# Autodesk Inventor assembly: body
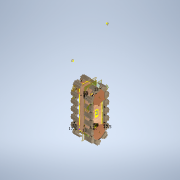
[picture p0: Inventor's stored thumbnail of the model, 180x180]
Saved by Autodesk Inventor 2020 (Build 240168000, 168)
## iProperties
Created: 2020-02-17
Part Number: body
Document SubType Name: Assembly
Designer: erwin
Author: erwin
## Documents named in this file (12)
- D:\GitHub\BeachMaid\platform-2\body.iam
- D:\GitHub\BeachMaid\platform-2\side.ipt
- D:\GitHub\BeachMaid\platform-2\middle.ipt
- D:\GitHub\BeachMaid\platform-2\internal.ipt
- D:\GitHub\BeachMaid\platform-2\cover.ipt
- D:\GitHub\BeachMaid\platform-2\plastic_lip.ipt
- D:\GitHub\BeachMaid\platform-2\spacer_battery_pack.ipt
- D:\GitHub\BeachMaid\platform-2\body\AIP\Tube and Pipe\Cable and Harness\body.Harness1.iam
- D:\GitHub\BeachMaid\platform\vent_cover.ipt
- D:\GitHub\BeachMaid\platform\motor_frontalholder.ipt
- D:\GitHub\BeachMaid\platform\sprocket7.ipt
- D:\GitHub\BeachMaid\platform-2\spacer_chain_link.ipt
## Components (22 placed, 11 different names)
1. side:1 — Flush:1, Flush:2, Flush:4, Rigid:2, Rotational:1, Rotational:4, Rotational:5
2. middle:1 — Flush:1, Flush:2, Mate:1, Flush:3, Flush:5, Flush:6, Flush:7, Flush:8, Mate:4, Mate:5, Planar:1, Planar:3, Planar:4
3. side:2 — Mate:1, Flush:3, Flush:4, Rigid:1, Rotational:2, Rotational:7, Rotational:6
4. internal:1 — Flush:5, Flush:6, Flush:11
5. cover:1 — Flush:7, Flush:8, Flush:9, Flush:10, Flush:11, Mate:2, Flush:12, Mate:3
6. plastic_lip:1 — Flush:9, Flush:10
7. plastic_lip:2 — Mate:2, Flush:12, Mate:3
8. internal:2 — Mate:4, Mate:5
9. spacer_battery_pack:1 — Planar:3
10. spacer_battery_pack:2 — Planar:4
11. spacer_battery_pack:3 — Planar:1
12. Harness1 [sub-assembly]
13. vent_cover:1 — Rigid:2
14. vent_cover:2 — Rigid:1
15. motor_frontalholder:1 — Rotational:2
16. motor_frontalholder:2 — Rotational:1
17. sprocket7:1 — Rotational:6
18. sprocket7:2 — Rotational:4
19. sprocket7:3 — Rotational:5
20. sprocket7:4 — Rotational:7
21. spacer_chain_link:1
22. spacer_chain_link:2
## Relationships (28: Flush 12, RevoluteJoint 6, Mate 5, PlanarJoint 3, WeldJoint 2)
- Flush:1: side:1 ↔ middle:1
- Flush:2: side:1 ↔ middle:1
- Mate:1: middle:1 ↔ side:2
- Flush:3: middle:1 ↔ side:2
- Flush:4: side:1 ↔ side:2
- Flush:5: middle:1 ↔ internal:1
- Flush:6: middle:1 ↔ internal:1
- Flush:7: middle:1 ↔ cover:1
- Flush:8: middle:1 ↔ cover:1
- Flush:9: cover:1 ↔ plastic_lip:1
- Flush:10: cover:1 ↔ plastic_lip:1
- Flush:11: internal:1 ↔ cover:1
- Mate:2: cover:1 ↔ plastic_lip:2
- Flush:12: cover:1 ↔ plastic_lip:2
- Mate:3: cover:1 ↔ plastic_lip:2
- Mate:4: middle:1 ↔ internal:2
- Mate:5: middle:1 ↔ internal:2
- Planar:1: middle:1 ↔ spacer_battery_pack:3
- Planar:3: middle:1 ↔ spacer_battery_pack:1
- Rigid:1 [WeldJoint]: side:2 ↔ vent_cover:2
- Rigid:2 [WeldJoint]: side:1 ↔ vent_cover:1
- Rotational:1 [RevoluteJoint]: side:1 ↔ motor_frontalholder:2
- Rotational:2 [RevoluteJoint]: side:2 ↔ motor_frontalholder:1
- Planar:4: middle:1 ↔ spacer_battery_pack:2
- Rotational:4 [RevoluteJoint] (30 mm): side:1 ↔ sprocket7:2
- Rotational:7 [RevoluteJoint] (30 mm): side:2 ↔ sprocket7:4
- Rotational:5 [RevoluteJoint] (-30 mm): side:1 ↔ sprocket7:3
- Rotational:6 [RevoluteJoint] (-30 mm): side:2 ↔ sprocket7:1
## Named parameters: angle = -92.44425 deg
